# Autodesk Inventor assembly: 분류대_적재함_ASSEMBLY
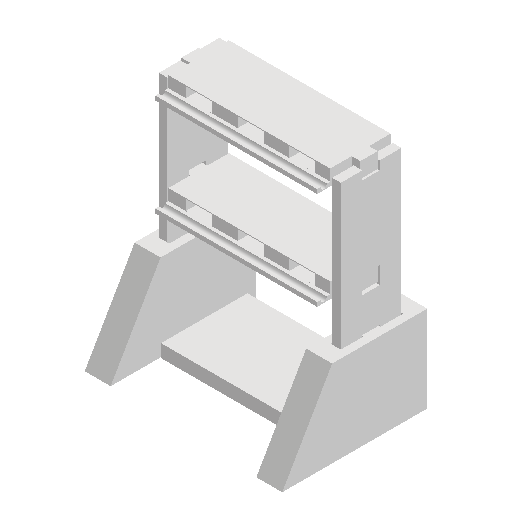
[picture p0: Inventor's stored thumbnail of the model, 512x512]
Saved by Autodesk Inventor 2027 (Build 310192000, 192)
## iProperties
Created: 2026-09-28
Part Number: 분류대_적재함_ASSEMBLY
Document SubType Name: Assembly
Designer: User
Author: User
## Documents named in this file (5)
- C:\Users\User\Desktop\4_권도영\졸업작품\INVENTOR\분류대_적재함\MAIN_분류대_적재함_ASSEMBLY.iam
- C:\Users\User\Desktop\4_권도영\졸업작품\INVENTOR\분류대_적재함\분류대_ASSEMBLY.iam
- C:\Users\User\Desktop\4_권도영\졸업작품\INVENTOR\분류대_적재함\적재함_부품_1.ipt
- C:\Users\User\Desktop\4_권도영\졸업작품\INVENTOR\분류대_적재함\적재함_부품_2.ipt
- C:\Users\User\Desktop\4_권도영\졸업작품\INVENTOR\분류대_적재함\적재함_브릿지.ipt
## Components (4 placed, 4 different names)
1. 분류대_ASSEMBLY:1 [sub-assembly] — 메이트:1, 메이트:2, 메이트:3, 메이트:4, 메이트:7, 메이트:8
2. 적재함_부품_1:1 — 메이트:1, 메이트:2, 메이트:5, 메이트:8
3. 적재함_부품_2:1 — 메이트:3, 메이트:4, 메이트:6, 메이트:7, 플러쉬:1
4. 적재함_브릿지:1 — 메이트:5, 메이트:6, 플러쉬:1
## Relationships (9: Mate 8, Flush 1)
- 메이트:1 [Mate]: 분류대_ASSEMBLY:1 ↔ 적재함_부품_1:1
- 메이트:2 [Mate]: 분류대_ASSEMBLY:1 ↔ 적재함_부품_1:1
- 메이트:3 [Mate]: 분류대_ASSEMBLY:1 ↔ 적재함_부품_2:1
- 메이트:4 [Mate]: 분류대_ASSEMBLY:1 ↔ 적재함_부품_2:1
- 메이트:5 [Mate]: 적재함_부품_1:1 ↔ 적재함_브릿지:1
- 메이트:6 [Mate]: 적재함_부품_2:1 ↔ 적재함_브릿지:1
- 메이트:7 [Mate]: 분류대_ASSEMBLY:1 ↔ 적재함_부품_2:1
- 메이트:8 [Mate]: 분류대_ASSEMBLY:1 ↔ 적재함_부품_1:1
- 플러쉬:1 [Flush]: 적재함_부품_2:1 ↔ 적재함_브릿지:1
